# Autodesk Inventor assembly: T-Copter
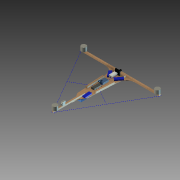
[picture p0: Inventor's stored thumbnail of the model, 180x180]
Saved by Autodesk Inventor 2013 SP1 (Build 170176100, 176)
## iProperties
Created: 2013-02-28
Part Number: T-Copter
Document SubType Name: Assembly
Designer: fixer
Mass: 817.762 g
Surface Area: 2773.81 cm^2
Volume: 743.837 cm^3
Density: 1.09938 g/cm^3
RuleStatus: InUse
Author: fixer
## Documents named in this file (22)
- D:\Users\fixer\Documents\Inventor\T-Copter\Design\T-Copter.iam
- D:\Users\fixer\Documents\Inventor\T-Copter\Design\Arm.ipt
- D:\Users\fixer\Documents\Inventor\T-Copter\Design\Rangelink Reciever.ipt
- D:\Users\fixer\Documents\Inventor\T-Copter\Design\Video Tx.ipt
- D:\Users\fixer\Documents\Inventor\T-Copter\Design\Lisa-M.ipt
- D:\Users\fixer\Documents\Inventor\T-Copter\Design\ESC - HK 20A.ipt
- D:\Users\fixer\Documents\Inventor\T-Copter\Design\Battery - 3S 2200mAh.ipt
- D:\Users\fixer\Documents\Inventor\T-Copter\Design\Rear Arm.ipt
- D:\Users\fixer\Documents\Inventor\T-Copter\Design\Triangle.ipt
- D:\Users\fixer\Documents\Inventor\T-Copter\Design\Camera - SONY CCD.ipt
- D:\Users\fixer\Documents\Inventor\T-Copter\Design\Top Plate.ipt
- D:\Users\fixer\Documents\Inventor\T-Copter\Design\Servo.ipt
- D:\Users\fixer\Documents\Inventor\T-Copter\Design\Front Spacer.ipt
- D:\Users\fixer\Documents\Inventor\T-Copter\Design\Side Spacer.ipt
- D:\Users\fixer\Documents\Inventor\T-Copter\Design\Bottom Plate v2.ipt
- D:\Users\fixer\Documents\Inventor\T-Copter\Design\Motor - DT750.ipt
- D:\Users\fixer\Documents\Inventor\T-Copter\Design\T-Copter\AIP\FEA\anidk4ps0.fins
- D:\Users\fixer\Documents\Inventor\T-Copter\Design\T-Copter\AIP\FEA\anidk4pts.fsat
- D:\Users\fixer\Documents\Inventor\T-Copter\Design\T-Copter\AIP\FEA\anidk4pxc.ftes
- D:\Users\fixer\Documents\Inventor\T-Copter\Design\T-Copter\AIP\FEA\anidk4wm8.fwiz
- D:\Users\fixer\Documents\Inventor\T-Copter\Design\T-Copter\AIP\FEA\anidk4wtc.fmsh
- D:\Users\fixer\Documents\Inventor\T-Copter\Design\T-Copter\AIP\FEA\anidk4wtd.fres
## Components (21 placed, 15 different names)
1. Triangle — Mate:18, Mate:19, Mate:20, Mate:45, Mate:46
2. Bottom Plate — Flush:5, Mate:8, Mate:10, Mate:11, Mate:12, Mate:15, Flush:11, Flush:12, Mate:29, Mate:32, Mate:33, Mate:34, Mate:35, Mate:36, Mate:37, Flush:14, Mate:41
3. Top Plate — Flush:13, Mate:40, Flush:14, Mate:42
4. Side Spacer:2 — Mate:33, Mate:34, Mate:36
5. Side Spacer:1 — Mate:32, Mate:35, Mate:37
6. Front Spacer:1 — Mate:29, Mate:30, Mate:31
7. Arm — Mate:4, Flush:12, Mate:20, Mate:30, Mate:43, Tangent:2
8. Arm:2 — Mate:5, Flush:11, Mate:19, Mate:44, Tangent:1
9. Rear Arm — Mate:3, Mate:18, Mate:27, Flush:15, Tangent:3
10. Rangelink Reciever — Mate:12
11. Video Tx — Mate:25, Mate:42
12. Lisa-M — Mate:11, Flush:39, Mate:47
13. Battery - 3S 2200mAh — Mate:24, Mate:41
14. ESC - HK 20A:1 — Mate:8
15. ESC - HK 20A:3 — Mate:10
16. ESC - HK 20A:4
17. Camera - SONY CCD — Mate:26
18. Servo — Mate:27, Mate:28
19. Motor - DT750:1 — Flush:15, Flush:16, Tangent:3
20. Motor - DT750:2 — Mate:43, Mate:45, Tangent:2
21. Motor - DT750:3 — Mate:44, Mate:46, Tangent:1
## Relationships (45: Mate 33, Flush 9, Tangent 3)
- Mate:3: Rear Arm
- Flush:5: Bottom Plate
- Mate:4: Arm
- Mate:5: Arm:2
- Flush:6 (6.35 mm)
- Mate:8: Bottom Plate ↔ ESC - HK 20A:1
- Mate:10: Bottom Plate ↔ ESC - HK 20A:3
- Mate:11: Bottom Plate ↔ Lisa-M
- Mate:12: Bottom Plate ↔ Rangelink Reciever
- Mate:15 (-6.35 mm): Bottom Plate
- Flush:11: Bottom Plate ↔ Arm:2
- Flush:12: Bottom Plate ↔ Arm
- Mate:18: Triangle ↔ Rear Arm
- Mate:19: Triangle ↔ Arm:2
- Mate:20: Triangle ↔ Arm
- Mate:24: Battery - 3S 2200mAh
- Mate:25: Video Tx
- Mate:26: Camera - SONY CCD
- Mate:27: Rear Arm ↔ Servo
- Mate:28: Servo
- Mate:29: Bottom Plate ↔ Front Spacer:1
- Mate:30: Front Spacer:1 ↔ Arm
- Mate:31: Front Spacer:1
- Mate:32: Bottom Plate ↔ Side Spacer:1
- Mate:33: Bottom Plate ↔ Side Spacer:2
- Mate:34: Bottom Plate ↔ Side Spacer:2
- Mate:35: Bottom Plate ↔ Side Spacer:1
- Mate:36: Bottom Plate ↔ Side Spacer:2
- Mate:37: Bottom Plate ↔ Side Spacer:1
- Flush:39: Lisa-M
- Flush:13: Top Plate
- Mate:40: Top Plate
- Flush:14: Bottom Plate ↔ Top Plate
- Mate:41: Bottom Plate ↔ Battery - 3S 2200mAh
- Mate:42: Top Plate ↔ Video Tx
- Flush:15: Rear Arm ↔ Motor - DT750:1
- Flush:16: Motor - DT750:1
- Mate:43: Arm ↔ Motor - DT750:2
- Mate:44: Arm:2 ↔ Motor - DT750:3
- Mate:45: Triangle ↔ Motor - DT750:2
- Mate:46: Triangle ↔ Motor - DT750:3
- Tangent:1: Arm:2 ↔ Motor - DT750:3
- Tangent:2: Arm ↔ Motor - DT750:2
- Tangent:3: Rear Arm ↔ Motor - DT750:1
- Mate:47: Lisa-M
## Named parameters: sa_0 = 7620
note: some values were not read from the file. Shown as the stored number, unit unknown: "sa_0".
